# Autodesk Inventor assembly: VolledigGeassembleerdv001
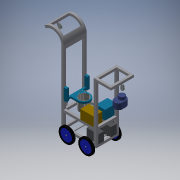
[picture p0: Inventor's stored thumbnail of the model, 180x180]
Saved by Autodesk Inventor 2017 (Build 210142000, 142)
## iProperties
Created: 2017-02-13
Part Number: VolledigGeassembleerdv001
Document SubType Name: Assembly
Designer: Koen
Author: Koen
## Documents named in this file (17)
- C:\Users\user\OneDrive\Inventor\VolledigGeassembleerdv001.iam
- C:\Users\user\OneDrive\Inventor\Frame.ipt
- C:\Users\user\OneDrive\Inventor\aandrijfMotor.ipt
- C:\Users\user\OneDrive\Inventor\asKogellager.ipt
- C:\Users\user\OneDrive\Inventor\as.ipt
- C:\Users\user\OneDrive\Inventor\wiel.ipt
- C:\Users\user\OneDrive\Inventor\kettingwiel.ipt
- C:\Users\user\OneDrive\Inventor\ketting1.ipt
- C:\Users\user\OneDrive\Inventor\ketting2.ipt
- C:\Users\user\OneDrive\Inventor\batterij.ipt
- C:\Users\user\OneDrive\Inventor\emmerhouder.ipt
- C:\Users\user\OneDrive\Inventor\emmer.ipt
- C:\Users\user\OneDrive\Inventor\winch.ipt
- C:\Users\user\OneDrive\Inventor\touw1.ipt
- C:\Users\user\OneDrive\Inventor\katrol.ipt
- C:\Users\user\OneDrive\Inventor\pomp.ipt
- C:\Users\user\OneDrive\Inventor\touw2.ipt
## Components (28 placed, 16 different names)
1. Frame:1 — Flush:1, Flush:6, Mate:13, Mate:14, Mate:15, Mate:16, Flush:12, Flush:13, Flush:14, Flush:15, Mate:19, Mate:20, Flush:18, Mate:26, Mate:27, Flush:21, Flush:22, Mate:28, Mate:29, Flush:23, Mate:31, Flush:24, Flush:25, Mate:34, Mate:35, Tangent:1, Flush:28, Mate:37, Mate:38, Flush:30, Tangent:3, Flush:32, Flush:33, Flush:36, Tangent:4, Mate:39
2. aandrijfMotor:1 — Flush:1, Flush:16, Flush:20, Flush:36
3. as:1 — Flush:6, Flush:7, Mate:9, Mate:11, Flush:8, Flush:11, Mate:22, Mate:23
4. as:2 — Flush:7, Mate:10, Mate:12, Flush:9, Flush:10, Mate:21, Mate:24, Mate:25
5. wiel:1 — Mate:9, Flush:8
6. wiel:2 — Mate:11, Flush:11
7. wiel:3 — Mate:12, Flush:10
8. wiel:4 — Mate:10, Flush:9
9. asKogellager:1 — Mate:16, Flush:15, Mate:18, Mate:19, Mate:22
10. asKogellager:2 — Mate:15, Flush:14, Mate:17, Mate:20, Mate:21
11. asKogellager:3 — Mate:14, Flush:13, Mate:17
12. asKogellager:4 — Mate:13, Flush:12, Mate:18
13. kettingwiel:1 — Mate:23, Flush:17, Flush:19
14. kettingwiel:2 — Mate:25, Flush:17, Flush:18
15. kettingwiel:3 — Mate:24, Flush:16
16. ketting1:1 — Flush:19
17. ketting2:1 — Flush:20
18. batterij:1 — Mate:26, Mate:27, Flush:21
19. batterij:2 — Flush:22, Mate:28, Mate:29
20. emmerhouder:1 — Flush:23, Mate:31, Flush:24, Insert:1
21. emmer:1 — Insert:1
22. winch:1 — Flush:25, Flush:27, Flush:29, Flush:34, Flush:35
23. touw1:1 — Flush:27, Flush:29
24. katrol:1 — Mate:34, Mate:35, Tangent:1
25. katrol:2 — Flush:28, Tangent:4, Mate:39
26. pomp:1 — Mate:37, Mate:38, Flush:30
27. katrol:3 — Tangent:3, Flush:32, Flush:33
28. touw2:1 — Flush:34, Flush:35
## Relationships (61: Flush 30, Mate 27, Tangent 3, Insert 1)
- Flush:1: Frame:1 ↔ aandrijfMotor:1
- Flush:6 (-50 mm): Frame:1 ↔ as:1
- Flush:7: as:1 ↔ as:2
- Mate:9: as:1 ↔ wiel:1
- Mate:10: as:2 ↔ wiel:4
- Mate:11: as:1 ↔ wiel:2
- Mate:12: as:2 ↔ wiel:3
- Flush:8: as:1 ↔ wiel:1
- Flush:9: as:2 ↔ wiel:4
- Flush:10: as:2 ↔ wiel:3
- Flush:11: as:1 ↔ wiel:2
- Mate:13: Frame:1 ↔ asKogellager:4
- Mate:14: Frame:1 ↔ asKogellager:3
- Mate:15: Frame:1 ↔ asKogellager:2
- Mate:16: Frame:1 ↔ asKogellager:1
- Flush:12: Frame:1 ↔ asKogellager:4
- Flush:13: Frame:1 ↔ asKogellager:3
- Flush:14: Frame:1 ↔ asKogellager:2
- Flush:15: Frame:1 ↔ asKogellager:1
- Mate:17: asKogellager:2 ↔ asKogellager:3
- Mate:18: asKogellager:1 ↔ asKogellager:4
- Mate:19 (-130 mm): Frame:1 ↔ asKogellager:1
- Mate:20 (-130 mm): Frame:1 ↔ asKogellager:2
- Mate:21: as:2 ↔ asKogellager:2
- Mate:22: as:1 ↔ asKogellager:1
- Mate:23: as:1 ↔ kettingwiel:1
- Mate:24: as:2 ↔ kettingwiel:3
- Mate:25: as:2 ↔ kettingwiel:2
- Flush:16: aandrijfMotor:1 ↔ kettingwiel:3
- Flush:17: kettingwiel:1 ↔ kettingwiel:2
- Flush:18 (-20 mm): Frame:1 ↔ kettingwiel:2
- Flush:19: kettingwiel:1 ↔ ketting1:1
- Flush:20: aandrijfMotor:1 ↔ ketting2:1
- Mate:26: Frame:1 ↔ batterij:1
- Mate:27: Frame:1 ↔ batterij:1
- Flush:21: Frame:1 ↔ batterij:1
- Flush:22: Frame:1 ↔ batterij:2
- Mate:28: Frame:1 ↔ batterij:2
- Mate:29: Frame:1 ↔ batterij:2
- Flush:23: Frame:1 ↔ emmerhouder:1
- Mate:31: Frame:1 ↔ emmerhouder:1
- Flush:24: Frame:1 ↔ emmerhouder:1
- Flush:25: Frame:1 ↔ winch:1
- Flush:27: winch:1 ↔ touw1:1
- Mate:34: Frame:1 ↔ katrol:1
- Mate:35 (25 mm): Frame:1 ↔ katrol:1
- Tangent:1: Frame:1 ↔ katrol:1
- Flush:28: Frame:1 ↔ katrol:2
- Flush:29: winch:1 ↔ touw1:1
- Mate:37 (150 mm): Frame:1 ↔ pomp:1
- Mate:38 (200 mm): Frame:1 ↔ pomp:1
- Flush:30: Frame:1 ↔ pomp:1
- Tangent:3: Frame:1 ↔ katrol:3
- Flush:32: Frame:1 ↔ katrol:3
- Flush:33: Frame:1 ↔ katrol:3
- Flush:34: winch:1 ↔ touw2:1
- Flush:35: winch:1 ↔ touw2:1
- Flush:36: Frame:1 ↔ aandrijfMotor:1
- Tangent:4: Frame:1 ↔ katrol:2
- Mate:39: Frame:1 ↔ katrol:2
- Insert:1: emmerhouder:1 ↔ emmer:1
